# Autodesk Inventor assembly: folivora
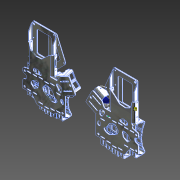
[picture p0: Inventor's stored thumbnail of the model, 180x180]
Saved by Autodesk Inventor 2018 (Build 220112000, 112)
## iProperties
Created: 2018-05-16
Part Number: folivora
Material: 一般
Document SubType Name: Assembly
Designer: NaMACHAN
Mass: 602.65 g
Surface Area: 2378.62 cm^2
Volume: 234.154 cm^3
Density: 2.57373 g/cm^3
Author: NaMACHAN
## Documents named in this file (26)
- C:\Users\NaMACHAN\Dropbox\Project\original\folivora\inventor\folivora.iam
- C:\Users\NaMACHAN\Dropbox\Project\original\folivora\inventor\baseframe.ipt
- C:\Users\NaMACHAN\Dropbox\Project\original\folivora\inventor\keyplate4.ipt
- C:\Users\NaMACHAN\Dropbox\Project\original\folivora\inventor\keyL.ipt
- C:\Users\NaMACHAN\Dropbox\Project\original\folivora\inventor\ball.ipt
- C:\Users\NaMACHAN\Dropbox\Project\original\folivora\inventor\trackball-base.ipt
- C:\Users\NaMACHAN\Dropbox\Project\original\folivora\inventor\trackball-shaft.ipt
- C:\Users\NaMACHAN\Dropbox\Project\original\folivora\inventor\bearing.ipt
- C:\Users\NaMACHAN\Dropbox\Project\original\folivora\inventor\bearingcover.ipt
- C:\Users\NaMACHAN\Dropbox\Project\original\folivora\inventor\trackball_l.ipt
- C:\Users\NaMACHAN\Dropbox\Project\original\folivora\inventor\trackball-cover.ipt
- C:\Users\NaMACHAN\Dropbox\Project\original\folivora\inventor\trackball-spacer.ipt
- C:\Users\NaMACHAN\Dropbox\Project\original\folivora\inventor\palmrest.ipt
- C:\Users\NaMACHAN\Dropbox\Project\original\folivora\inventor\palmrest-plate.ipt
- C:\Users\NaMACHAN\Dropbox\Project\original\folivora\inventor\baseframe_left.ipt
- C:\Users\NaMACHAN\Dropbox\Project\original\folivora\inventor\palmrest_left.ipt
- C:\Users\NaMACHAN\Dropbox\Project\original\folivora\inventor\thumbkey_L.ipt
- C:\Users\NaMACHAN\Dropbox\Project\original\folivora\inventor\keyplate2.ipt
- C:\Users\NaMACHAN\Dropbox\Project\original\folivora\inventor\keyplate5.ipt
- C:\Users\NaMACHAN\Dropbox\Project\original\folivora\inventor\keyL_extended.ipt
- C:\Users\NaMACHAN\Dropbox\Project\original\folivora\inventor\folivora\AIP\FEA\cjjue1qww.fins
- C:\Users\NaMACHAN\Dropbox\Project\original\folivora\inventor\folivora\AIP\FEA\cjjue1qww.fsat
- C:\Users\NaMACHAN\Dropbox\Project\original\folivora\inventor\folivora\AIP\FEA\cjjue1qww.ftes
- C:\Users\NaMACHAN\Dropbox\Project\original\folivora\inventor\folivora\AIP\FEA\cjjue1qww.fwiz
- C:\Users\NaMACHAN\Dropbox\Project\original\folivora\inventor\folivora\AIP\FEA\cjjue1r1c.fmsh
- C:\Users\NaMACHAN\Dropbox\Project\original\folivora\inventor\folivora\AIP\FEA\cjjue1r1d.fres
## Components (61 placed, 19 different names)
1. baseframe:1 — メイト:114, フラッシュ:19, フラッシュ:20, フラッシュ:23, フラッシュ:24, メイト:141, メイト:205, メイト:206, メイト:207, メイト:302, フラッシュ:57, フラッシュ:58
2. ball:1 — メイト:105, メイト:115
3. trackball-base:1 — メイト:52, メイト:53, メイト:54, メイト:55, メイト:56, メイト:57, メイト:58, メイト:59, メイト:60, メイト:61, メイト:62, メイト:63, フラッシュ:15, メイト:105, フラッシュ:16, メイト:117, メイト:118, メイト:119, メイト:120, メイト:124, メイト:125
4. trackball-shaft:1 — メイト:49, メイト:52, メイト:53, メイト:54
5. bearing:1 — メイト:49, メイト:55
6. trackball-shaft:2 — メイト:56, メイト:57, メイト:59
7. bearing:2 — メイト:58
8. trackball-shaft:3 — メイト:60, メイト:61, メイト:62
9. bearing:3 — メイト:63
10. bearingcover:1 — フラッシュ:15, フラッシュ:16, メイト:115, メイト:121, メイト:122, メイト:123, メイト:124, メイト:125, メイト:134, メイト:135, メイト:136
11. trackball_l:1 — メイト:114, メイト:121, メイト:122, メイト:123, フラッシュ:19, フラッシュ:20
12. trackball-shaft:4 — メイト:116, メイト:117, メイト:118, メイト:119
13. bearing:4 — メイト:116, メイト:120
14. trackball-cover:1 — メイト:126, メイト:127, メイト:128, メイト:129, メイト:130, メイト:131, メイト:132, メイト:133
15. trackball-spacer:1 — メイト:126, メイト:130, メイト:136
16. trackball-spacer:2 — メイト:129, メイト:131, メイト:135
17. trackball-spacer:3 — メイト:128, メイト:133
18. trackball-spacer:4 — メイト:127, メイト:132, メイト:134
19. palmrest:1 — メイト:205, メイト:206, メイト:207, メイト:209, メイト:210, メイト:217
20. baseframe_left:1 — フラッシュ:23, フラッシュ:24, メイト:141, メイト:189, メイト:190, メイト:191, メイト:192, メイト:201, フラッシュ:32, フラッシュ:33, メイト:214, メイト:215, メイト:216, メイト:223, フラッシュ:34, フラッシュ:35, メイト:236, メイト:240, メイト:245, メイト:253, メイト:259, メイト:262, メイト:263
21. palmrest_left:1 — メイト:211, メイト:212, メイト:213, メイト:214, メイト:215, メイト:216
22. keyL:16 — メイト:189, メイト:231, メイト:232, 角度:19, メイト:243
23. keyL:22 — メイト:192, メイト:229, メイト:230
24. keyL:24 — メイト:190, メイト:219, メイト:220, 角度:18, メイト:224
25. keyL:27 — メイト:191, メイト:227, メイト:228, 角度:20, メイト:238
26. thumbkey_L:1 — メイト:201, フラッシュ:32, フラッシュ:33, メイト:202, メイト:203, メイト:218
27. keyplate2:1 — メイト:202, メイト:203, メイト:218
28. palmrest-plate:1 — メイト:209, メイト:210, メイト:217
29. palmrest-plate:2 — メイト:211, メイト:212, メイト:213
30. keyplate5:1 — メイト:231, メイト:232, 角度:19, メイト:243, メイト:244, メイト:246, メイト:247, メイト:260
31. keyL_extended:1 — メイト:221, メイト:222, メイト:223, フラッシュ:34, フラッシュ:35, フラッシュ:36
32. keyplate4:7 — メイト:219, メイト:220, メイト:221, メイト:222, 角度:18, メイト:224, メイト:235
33. keyplate5:2 — メイト:227, メイト:228, 角度:20, メイト:238, メイト:239, メイト:241, メイト:242, メイト:247
34. keyplate5:3 — メイト:229, メイト:230, メイト:233, メイト:234, メイト:235, メイト:237, メイト:239
35. keyL_extended:2 — メイト:233, メイト:234, フラッシュ:36, メイト:236, メイト:237, フラッシュ:37
36. keyL_extended:3 — メイト:240, メイト:241, メイト:242, フラッシュ:37, フラッシュ:38
37. keyL_extended:4 — メイト:244, メイト:245, メイト:246, フラッシュ:38, フラッシュ:39
38. keyL:28 — メイト:253
39. keyL_extended:5 — メイト:263, フラッシュ:39, フラッシュ:40
40. keyplate4:8 — メイト:260, メイト:261
41. keyL:29 — メイト:259
42. keyL_extended:6 — メイト:262, フラッシュ:40
43. keyplate4:9 — メイト:261
44. keyL:30 — フラッシュ:52, フラッシュ:53
45. keyL:31 — フラッシュ:54, フラッシュ:55
46. keyL:32 — フラッシュ:55
47. keyL:33 — フラッシュ:53, フラッシュ:54
48. keyplate5:4 — メイト:298, メイト:299
49. keyL_extended:7 — フラッシュ:50, フラッシュ:58
50. keyplate4:10 — メイト:301
51. keyplate5:5 — メイト:299, メイト:300
52. keyplate5:6 — メイト:300, メイト:301
53. keyL_extended:8 — フラッシュ:49, フラッシュ:50
54. keyL_extended:9 — フラッシュ:47, フラッシュ:49, フラッシュ:57
55. keyL_extended:10 — フラッシュ:47, フラッシュ:48
56. keyL:34 — フラッシュ:51, フラッシュ:52
57. keyL_extended:11 — フラッシュ:46, フラッシュ:48, フラッシュ:56
58. keyplate4:11 — メイト:297, メイト:298
59. keyL:35 — フラッシュ:51, フラッシュ:56
60. keyL_extended:12 — フラッシュ:46, メイト:302
61. keyplate4:12 — メイト:297
## Relationships (182: Mate 139, Flush 33, Angle 10)
- メイト:49 [Mate]: trackball-shaft:1 ↔ bearing:1
- [Mate]: trackball-shaft:2 ↔ bearing:2
- [Mate]: trackball-shaft:3 ↔ bearing:3
- メイト:52 [Mate] (1.5 mm): trackball-base:1 ↔ trackball-shaft:1
- メイト:53 [Mate] (1.5 mm): trackball-base:1 ↔ trackball-shaft:1
- メイト:54 [Mate]: trackball-base:1 ↔ trackball-shaft:1
- メイト:55 [Mate] (0.5 mm): trackball-base:1 ↔ bearing:1
- メイト:56 [Mate] (1.5 mm): trackball-base:1 ↔ trackball-shaft:2
- メイト:57 [Mate] (1.5 mm): trackball-base:1 ↔ trackball-shaft:2
- メイト:58 [Mate] (0.5 mm): trackball-base:1 ↔ bearing:2
- メイト:59 [Mate]: trackball-base:1 ↔ trackball-shaft:2
- メイト:60 [Mate] (1.5 mm): trackball-base:1 ↔ trackball-shaft:3
- メイト:61 [Mate] (1.5 mm): trackball-base:1 ↔ trackball-shaft:3
- メイト:62 [Mate]: trackball-base:1 ↔ trackball-shaft:3
- メイト:63 [Mate] (0.5 mm): trackball-base:1 ↔ bearing:3
- フラッシュ:15 [Flush]: trackball-base:1 ↔ bearingcover:1
- メイト:105 [Mate]: ball:1 ↔ trackball-base:1
- メイト:114 [Mate]: baseframe:1 ↔ trackball_l:1
- フラッシュ:16 [Flush]: trackball-base:1 ↔ bearingcover:1
- メイト:115 [Mate] (6.4 mm): ball:1 ↔ bearingcover:1
- メイト:116 [Mate]: trackball-shaft:4 ↔ bearing:4
- メイト:117 [Mate] (1.5 mm): trackball-base:1 ↔ trackball-shaft:4
- メイト:118 [Mate] (1.5 mm): trackball-base:1 ↔ trackball-shaft:4
- メイト:119 [Mate]: trackball-base:1 ↔ trackball-shaft:4
- メイト:120 [Mate] (0.5 mm): trackball-base:1 ↔ bearing:4
- メイト:121 [Mate]: bearingcover:1 ↔ trackball_l:1
- メイト:122 [Mate]: bearingcover:1 ↔ trackball_l:1
- メイト:123 [Mate]: bearingcover:1 ↔ trackball_l:1
- メイト:124 [Mate]: trackball-base:1 ↔ bearingcover:1
- メイト:125 [Mate]: trackball-base:1 ↔ bearingcover:1
- メイト:126 [Mate]: trackball-cover:1 ↔ trackball-spacer:1
- メイト:127 [Mate]: trackball-cover:1 ↔ trackball-spacer:4
- メイト:128 [Mate]: trackball-cover:1 ↔ trackball-spacer:3
- メイト:129 [Mate]: trackball-cover:1 ↔ trackball-spacer:2
- メイト:130 [Mate]: trackball-cover:1 ↔ trackball-spacer:1
- メイト:131 [Mate]: trackball-cover:1 ↔ trackball-spacer:2
- メイト:132 [Mate]: trackball-cover:1 ↔ trackball-spacer:4
- メイト:133 [Mate]: trackball-cover:1 ↔ trackball-spacer:3
- メイト:134 [Mate]: bearingcover:1 ↔ trackball-spacer:4
- メイト:135 [Mate]: bearingcover:1 ↔ trackball-spacer:2
- メイト:136 [Mate]: bearingcover:1 ↔ trackball-spacer:1
- フラッシュ:19 [Flush] (-10 mm): baseframe:1 ↔ trackball_l:1
- フラッシュ:20 [Flush] (-10 mm): baseframe:1 ↔ trackball_l:1
- フラッシュ:23 [Flush]: baseframe:1 ↔ baseframe_left:1
- フラッシュ:24 [Flush]: baseframe:1 ↔ baseframe_left:1
- メイト:141 [Mate] (100 mm): baseframe:1 ↔ baseframe_left:1
- メイト:189 [Mate]: baseframe_left:1 ↔ keyL:16
- メイト:190 [Mate]: baseframe_left:1 ↔ keyL:24
- メイト:191 [Mate]: baseframe_left:1 ↔ keyL:27
- メイト:192 [Mate]: baseframe_left:1 ↔ keyL:22
- メイト:201 [Mate]: baseframe_left:1 ↔ thumbkey_L:1
- フラッシュ:32 [Flush] (12 mm): baseframe_left:1 ↔ thumbkey_L:1
- フラッシュ:33 [Flush]: baseframe_left:1 ↔ thumbkey_L:1
- メイト:202 [Mate]: thumbkey_L:1 ↔ keyplate2:1
- メイト:203 [Mate]: thumbkey_L:1 ↔ keyplate2:1
- メイト:205 [Mate]: baseframe:1 ↔ palmrest:1
- メイト:206 [Mate]: baseframe:1 ↔ palmrest:1
- メイト:207 [Mate]: baseframe:1 ↔ palmrest:1
- メイト:209 [Mate]: palmrest:1 ↔ palmrest-plate:1
- メイト:210 [Mate]: palmrest:1 ↔ palmrest-plate:1
- メイト:211 [Mate]: palmrest_left:1 ↔ palmrest-plate:2
- メイト:212 [Mate]: palmrest_left:1 ↔ palmrest-plate:2
- メイト:213 [Mate]: palmrest_left:1 ↔ palmrest-plate:2
- メイト:214 [Mate]: baseframe_left:1 ↔ palmrest_left:1
- メイト:215 [Mate]: baseframe_left:1 ↔ palmrest_left:1
- メイト:216 [Mate]: baseframe_left:1 ↔ palmrest_left:1
- メイト:217 [Mate]: palmrest:1 ↔ palmrest-plate:1
- メイト:218 [Mate]: thumbkey_L:1 ↔ keyplate2:1
- メイト:219 [Mate] (1.5 mm): keyL:24 ↔ keyplate4:7
- メイト:220 [Mate]: keyL:24 ↔ keyplate4:7
- メイト:221 [Mate]: keyL_extended:1 ↔ keyplate4:7
- メイト:222 [Mate] (1.5 mm): keyL_extended:1 ↔ keyplate4:7
- メイト:223 [Mate]: baseframe_left:1 ↔ keyL_extended:1
- 角度:18 [Angle] (0 deg): keyL:24 ↔ keyplate4:7
- メイト:224 [Mate] (15 mm): keyL:24 ↔ keyplate4:7
- メイト:227 [Mate] (1.5 mm): keyL:27 ↔ keyplate5:2
- メイト:228 [Mate]: keyL:27 ↔ keyplate5:2
- メイト:229 [Mate]: keyL:22 ↔ keyplate5:3
- メイト:230 [Mate] (1.5 mm): keyL:22 ↔ keyplate5:3
- メイト:231 [Mate]: keyL:16 ↔ keyplate5:1
- メイト:232 [Mate]: keyL:16 ↔ keyplate5:1
- 角度:19 [Angle] (0 deg): keyL:16 ↔ keyplate5:1
- 角度:20 [Angle] (0 deg): keyL:27 ↔ keyplate5:2
- フラッシュ:34 [Flush] (-20 mm): baseframe_left:1 ↔ keyL_extended:1
- フラッシュ:35 [Flush] (13 mm): baseframe_left:1 ↔ keyL_extended:1
- メイト:233 [Mate] (1.5 mm): keyplate5:3 ↔ keyL_extended:2
- メイト:234 [Mate]: keyplate5:3 ↔ keyL_extended:2
- フラッシュ:36 [Flush] (3 mm): keyL_extended:1 ↔ keyL_extended:2
- メイト:235 [Mate]: keyplate4:7 ↔ keyplate5:3
- メイト:236 [Mate]: baseframe_left:1 ↔ keyL_extended:2
- メイト:237 [Mate] (17 mm): keyplate5:3 ↔ keyL_extended:2
- メイト:238 [Mate] (15 mm): keyL:27 ↔ keyplate5:2
- メイト:239 [Mate]: keyplate5:2 ↔ keyplate5:3
- メイト:240 [Mate]: baseframe_left:1 ↔ keyL_extended:3
- メイト:241 [Mate] (1.5 mm): keyplate5:2 ↔ keyL_extended:3
- メイト:242 [Mate]: keyplate5:2 ↔ keyL_extended:3
- フラッシュ:37 [Flush] (-3 mm): keyL_extended:2 ↔ keyL_extended:3
- メイト:243 [Mate] (13 mm): keyL:16 ↔ keyplate5:1
- メイト:244 [Mate] (1.5 mm): keyplate5:1 ↔ keyL_extended:4
- メイト:245 [Mate]: baseframe_left:1 ↔ keyL_extended:4
- メイト:246 [Mate]: keyplate5:1 ↔ keyL_extended:4
- フラッシュ:38 [Flush] (3 mm): keyL_extended:3 ↔ keyL_extended:4
- メイト:247 [Mate]: keyplate5:1 ↔ keyplate5:2
- [Mate] (1.5 mm): keyL:28 ↔ keyplate4:8
- [Mate]: keyL:28 ↔ keyplate4:8
- [Mate]: keyL_extended:5 ↔ keyplate4:8
- [Mate] (1.5 mm): keyL_extended:5 ↔ keyplate4:8
- [Angle] (0 deg): keyL:28 ↔ keyplate4:8
- [Mate] (15 mm): keyL:28 ↔ keyplate4:8
- メイト:253 [Mate]: baseframe_left:1 ↔ keyL:28
- [Mate] (1.5 mm): keyL:29 ↔ keyplate4:9
- [Mate]: keyL:29 ↔ keyplate4:9
- [Mate]: keyL_extended:6 ↔ keyplate4:9
- [Mate] (1.5 mm): keyL_extended:6 ↔ keyplate4:9
- [Angle] (0 deg): keyL:29 ↔ keyplate4:9
- [Mate] (15 mm): keyL:29 ↔ keyplate4:9
- メイト:259 [Mate]: baseframe_left:1 ↔ keyL:29
- メイト:260 [Mate]: keyplate5:1 ↔ keyplate4:8
- メイト:261 [Mate]: keyplate4:8 ↔ keyplate4:9
- メイト:262 [Mate]: baseframe_left:1 ↔ keyL_extended:6
- メイト:263 [Mate]: baseframe_left:1 ↔ keyL_extended:5
- フラッシュ:39 [Flush] (-20 mm): keyL_extended:4 ↔ keyL_extended:5
- フラッシュ:40 [Flush] (1 mm): keyL_extended:5 ↔ keyL_extended:6
- [Mate] (1.5 mm): keyL:32 ↔ keyplate4:10
- [Mate]: keyL:32 ↔ keyplate4:10
- [Mate]: keyL_extended:7 ↔ keyplate4:10
- [Mate] (1.5 mm): keyL_extended:7 ↔ keyplate4:10
- [Angle] (0 deg): keyL:32 ↔ keyplate4:10
- [Mate] (15 mm): keyL:32 ↔ keyplate4:10
- [Mate] (1.5 mm): keyL:33 ↔ keyplate5:5
- [Mate]: keyL:33 ↔ keyplate5:5
- [Mate]: keyL:31 ↔ keyplate5:6
- [Mate] (1.5 mm): keyL:31 ↔ keyplate5:6
- [Mate]: keyL:30 ↔ keyplate5:4
- [Mate]: keyL:30 ↔ keyplate5:4
- [Angle] (0 deg): keyL:30 ↔ keyplate5:4
- [Angle] (0 deg): keyL:33 ↔ keyplate5:5
- [Mate] (1.5 mm): keyplate5:6 ↔ keyL_extended:8
- [Mate]: keyplate5:6 ↔ keyL_extended:8
- [Flush] (3 mm): keyL_extended:7 ↔ keyL_extended:8
- [Mate] (17 mm): keyplate5:6 ↔ keyL_extended:8
- [Mate] (15 mm): keyL:33 ↔ keyplate5:5
- [Mate] (1.5 mm): keyplate5:5 ↔ keyL_extended:9
- [Mate]: keyplate5:5 ↔ keyL_extended:9
- [Flush] (-3 mm): keyL_extended:8 ↔ keyL_extended:9
- [Mate] (13 mm): keyL:30 ↔ keyplate5:4
- [Mate] (1.5 mm): keyplate5:4 ↔ keyL_extended:10
- [Mate]: keyplate5:4 ↔ keyL_extended:10
- [Flush] (3 mm): keyL_extended:9 ↔ keyL_extended:10
- [Mate] (1.5 mm): keyL:34 ↔ keyplate4:11
- [Mate]: keyL:34 ↔ keyplate4:11
- [Mate]: keyL_extended:11 ↔ keyplate4:11
- [Mate] (1.5 mm): keyL_extended:11 ↔ keyplate4:11
- [Angle] (0 deg): keyL:34 ↔ keyplate4:11
- [Mate] (15 mm): keyL:34 ↔ keyplate4:11
- [Mate] (1.5 mm): keyL:35 ↔ keyplate4:12
- [Mate]: keyL:35 ↔ keyplate4:12
- [Mate]: keyL_extended:12 ↔ keyplate4:12
- [Mate] (1.5 mm): keyL_extended:12 ↔ keyplate4:12
- [Angle] (0 deg): keyL:35 ↔ keyplate4:12
- [Mate] (15 mm): keyL:35 ↔ keyplate4:12
- [Flush] (-20 mm): keyL_extended:10 ↔ keyL_extended:11
- [Flush] (1 mm): keyL_extended:11 ↔ keyL_extended:12
- フラッシュ:46 [Flush]: keyL_extended:11 ↔ keyL_extended:12
- フラッシュ:47 [Flush]: keyL_extended:9 ↔ keyL_extended:10
- フラッシュ:48 [Flush]: keyL_extended:10 ↔ keyL_extended:11
- フラッシュ:49 [Flush]: keyL_extended:8 ↔ keyL_extended:9
- フラッシュ:50 [Flush]: keyL_extended:7 ↔ keyL_extended:8
- フラッシュ:51 [Flush]: keyL:34 ↔ keyL:35
- フラッシュ:52 [Flush]: keyL:30 ↔ keyL:34
- フラッシュ:53 [Flush]: keyL:30 ↔ keyL:33
- フラッシュ:54 [Flush]: keyL:31 ↔ keyL:33
- フラッシュ:55 [Flush]: keyL:31 ↔ keyL:32
- フラッシュ:56 [Flush]: keyL_extended:11 ↔ keyL:35
- メイト:297 [Mate]: keyplate4:11 ↔ keyplate4:12
- メイト:298 [Mate]: keyplate5:4 ↔ keyplate4:11
- メイト:299 [Mate]: keyplate5:4 ↔ keyplate5:5
- メイト:300 [Mate]: keyplate5:5 ↔ keyplate5:6
- メイト:301 [Mate]: keyplate4:10 ↔ keyplate5:6
- メイト:302 [Mate]: baseframe:1 ↔ keyL_extended:12
- フラッシュ:57 [Flush] (-20 mm): baseframe:1 ↔ keyL_extended:9
- フラッシュ:58 [Flush] (13 mm): baseframe:1 ↔ keyL_extended:7
## Named parameters: sa_0 = 7.4e-12, sa_1 = -5000, sa_2 = 4e-13, sa_3 = -1.32e-11, sa_4 = -5000, sa_5 = -4.2e-12, sa_6 = -2.8e-12, sa_7 = -5000, sa_8 = -2.3e-12, sa_9 = -1e-12, sa_10 = -5000, sa_11 = -3.7e-12, sa_12 = 2.78e-11, sa_13 = -5000, sa_14 = 7e-12, sa_15 = 1.85e-11, sa_16 = -5000, sa_17 = 3.9e-12, d430_d429 = 0 mm, d431_d429 = 0 mm, d833_d799 = 1.5 mm, d834_d801 = 0 deg, d835_d802 = 15 mm, d836_d796 = 1.5 mm, d837_d797 = 0 mm, d838_d798 = 0 mm, d840_d799 = 1.5 mm, d841_d801 = 0 deg, d842_d802 = 15 mm, d843_d796 = 1.5 mm, d844_d797 = 0 mm, d845_d798 = 0 mm, d855_d851 = -20 mm, d856_d852 = 1 mm, d857_d826 = -3 mm, d858_d827 = 13 mm, d859_d828 = 1.5 mm, d860_d830 = 0 mm, d861_d831 = 3 mm, d863_d833_d799 = 1.5 mm, d864_d834_d801 = 0 deg, d865_d835_d802 = 15 mm, d866_d836_d796 = 1.5 mm, d867_d837_d797 = 0 mm, d868_d838_d798 = 0 mm, d869_d840_d799 = 1.5 mm, d870_d841_d801 = 0 deg, d871_d842_d802 = 15 mm, d872_d843_d796 = 1.5 mm, d873_d844_d797 = 0 mm, d874_d845_d798 = 0 mm, d875_d817 = 3 mm, d877_d820 = 17 mm, d878_d821 = 15 mm, d880_d824 = 1.5 mm, d881_d825 = 0 mm, d882_d808 = 1.5 mm, d883_d809 = 0 mm, d884_d810 = 0 mm, d885_d811 = 0 deg, d886_d812 = 0 deg, d887_d815 = 1.5 mm, d888_d816 = 0 mm, d889_d799 = 1.5 mm, d890_d801 = 0 deg, d891_d802 = 15 mm, d892_d805 = 1.5 mm, d893_d806 = 0 mm, d894_d807 = 0 mm, d895_d796 = 1.5 mm, d896_d797 = 0 mm, d897_d798 = 0 mm
note: some values were not read from the file. Shown as the stored number, unit unknown: "sa_0", "sa_1", "sa_2", "sa_3", "sa_4", "sa_5", "sa_6", "sa_7", "sa_8", "sa_9", "sa_10", "sa_11", "sa_12", "sa_13", "sa_14", "sa_15", "sa_16", "sa_17".
